# Autodesk Inventor assembly: 右足アセンブリ_MIR
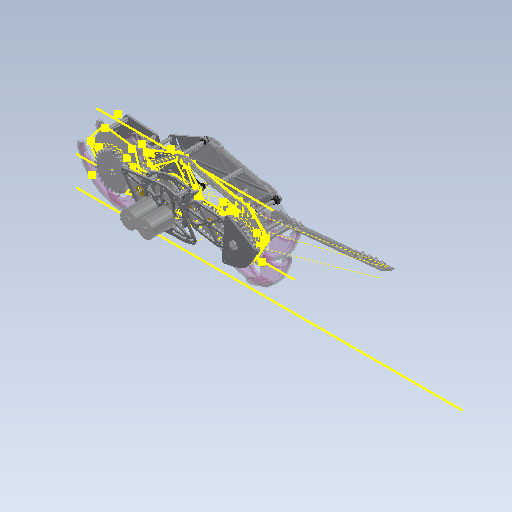
[picture p0: Inventor's stored thumbnail of the model, 512x512]
Saved by Autodesk Inventor 2020 (Build 240168000, 168)
## iProperties
Created: 2019-09-17
Part Number: 右足アセンブリ_MIR
Material: 一般
Document SubType Name: Assembly
Designer: tanjihayato
Mass: 648.248 g
Surface Area: 3194.36 cm^2
Volume: 323.123 cm^3
Density: 2.00619 g/cm^3
Author: tanjihayato
## Documents named in this file (44)
- \\Mac\Home\Documents\Inventor\2019お遊び機体\右足アセンブリ_MIR.iam
- \\Mac\Home\Documents\Inventor\2019お遊び機体\前足内フレーム_MIR1.ipt
- \\Mac\Home\Documents\Inventor\2019お遊び機体\新型３クランクアセンブリ_MIR2.iam
- \\Mac\Home\Documents\Inventor\2019お遊び機体\新型３脚最終段カム.ipt
- \\Mac\Home\Documents\Inventor\2019お遊び機体\スペーサ　m3-l35.ipt
- \\Mac\Home\Documents\Inventor\2019お遊び機体\新型３ヘッケン_MIR2.ipt
- \\Mac\Home\Documents\Inventor\2019お遊び機体\新型３揺動節_MIR2.ipt
- \\Mac\Home\Documents\Inventor\2019お遊び機体\線図_MIR.ipt
- \\Mac\Home\Documents\Inventor\2019お遊び機体\ギアトレイン_MIR1.ipt
- \\Mac\Home\Documents\Inventor\2019お遊び機体\スペーサ　m3-l6.ipt
- \\Mac\Home\Documents\Inventor\2019お遊び機体\前足外フレーム_MIR1.ipt
- \\Mac\Home\Documents\Inventor\2019お遊び機体\後ろ脚内フレーム_MIR1.ipt
- \\Mac\Home\Documents\Inventor\2019お遊び機体\後ろ脚内フレーム２_MIR1.ipt
- \\Mac\Home\Documents\Inventor\2019お遊び機体\新型３クランクアセンブリ_MIR_MIR1.iam
- \\Mac\Home\Documents\Inventor\2019お遊び機体\新型３ヘッケン_MIR_MIR1.ipt
- \\Mac\Home\Documents\Inventor\2019お遊び機体\新型３揺動節_MIR_MIR1.ipt
- \\Mac\Home\Documents\Inventor\2019お遊び機体\後ろ脚外フレーム_MIR1.ipt
- \\Mac\Home\Documents\Inventor\2019お遊び機体\前足ギアトレイン抑え_MIR.ipt
- \\Mac\Home\Documents\Inventor\2019お遊び機体\スペーサ　m3-l12.ipt
- \\Mac\Home\Documents\Inventor\2019お遊び機体\新型３脚最終段カム2.ipt
- \\Mac\Home\Documents\Inventor\2019お遊び機体\z28ギア(インベンター).ipt
- \\Mac\Home\Documents\Inventor\2019お遊び機体\z20ギア(インベンター).ipt
- \\Mac\Home\Documents\Inventor\2019お遊び機体\ベアリングフランジ6-12.ipt
- \\Mac\Home\Documents\Inventor\2019お遊び機体\z17ギア(インベンター).ipt
- \\Mac\Home\Documents\Inventor\2019お遊び機体\中間内フレーム2_MIR.ipt
- \\Mac\Home\Documents\Inventor\2019お遊び機体\サス軸抑え外_MIR.ipt
- \\Mac\Home\Documents\Inventor\2019お遊び機体\中間外フレーム2_MIR.ipt
- \\Mac\Home\Documents\Inventor\2019お遊び機体\スペーサ　m3-l3.ipt
- \\Mac\Home\Documents\Inventor\2019お遊び機体\タミヤダンパー1.iam
- \\Mac\Home\Documents\Inventor\2019お遊び機体\脚ゴム_MIR.ipt
- \\Mac\Home\Documents\Inventor\2019お遊び機体\歯車m0.5.z80.ipt
- \\Mac\Home\Documents\Inventor\2019お遊び機体\m2z10.ipt
- \\Mac\Home\Documents\Inventor\2019お遊び機体\中間フレーム内内_MIR.ipt
- \\Mac\Home\Documents\Inventor\2019お遊び機体\モーター(形だけ).ipt
- \\Mac\Home\Documents\Inventor\2019お遊び機体\スペーサ　m3-l20.ipt
- \\Mac\Home\Documents\Inventor\2019お遊び機体\脚モーターマウント_MIR.ipt
- \\Mac\Home\Documents\Inventor\2019お遊び機体\台形サスバー２.ipt
- \\Mac\Home\Documents\Inventor\2019お遊び機体\フランジブッシュ　d6-D8-l5-h12.ipt
- \\Mac\Home\Documents\Inventor\2019お遊び機体\スペーサ　m3-l45.ipt
- \\Mac\Home\Documents\Inventor\2019お遊び機体\台形サスバー板.ipt
- \\Mac\Home\Documents\Inventor\2019お遊び機体\台形サスカバー_MIR.ipt
- \\Mac\Home\Documents\Inventor\2019お遊び機体\カウンター短.ipt
- \\Mac\Home\Documents\Inventor\2019お遊び機体\ベアリングH　d6-D10-B3.ipt
- \\Mac\Home\Documents\Inventor\2019お遊び機体\スペーサ　m4-l35.ipt
## Components (114 placed, 43 different names)
1. 前足内フレーム_MIR1:1 — 挿入:29, 挿入:32, 挿入:37, 挿入:59, 挿入:61, 挿入:126, 挿入:127, 挿入:135, 挿入:134, 挿入:107, 挿入:108
2. 新型３クランクアセンブリ_MIR2:1 [sub-assembly] — メイト:1, 挿入:1, 挿入:11, 挿入:10, 挿入:9, 挿入:8
3. 新型３脚最終段カム:1 — メイト:1, 挿入:1, メイト:44, 挿入:62, 挿入:107
4. スペーサ　m3-l35:1 — 挿入:29
5. スペーサ　m3-l35:2 — 挿入:32, メイト:2, メイト:3, メイト:4, メイト:5, メイト:15
6. 新型３ヘッケン_MIR2:1 — 挿入:11, 挿入:14, フラッシュ:2, メイト:57, メイト:56
7. 新型３ヘッケン_MIR2:2 — 挿入:10, 挿入:13, フラッシュ:4, メイト:61, メイト:60
8. 新型３ヘッケン_MIR2:3 — 挿入:9, 挿入:12, フラッシュ:5, メイト:63, メイト:62
9. 新型３ヘッケン_MIR2:4 — 挿入:8, 挿入:7, フラッシュ:3, メイト:59, メイト:58
10. 新型３揺動節_MIR2:1 — 挿入:7, メイト:2
11. 新型３揺動節_MIR2:2 — 挿入:13, メイト:3
12. 新型３揺動節_MIR2:3 — 挿入:12, メイト:4
13. 新型３揺動節_MIR2:4 — 挿入:14, メイト:5
14. 線図_MIR:1 — メイト:51
15. ギアトレイン_MIR1:1 — 挿入:17, 挿入:20, 挿入:19, 挿入:16, 挿入:15, 挿入:18, 挿入:103
16. ギアトレイン_MIR1:2 — 挿入:37, メイト:10, 挿入:21
17. スペーサ　m3-l6:1 — 挿入:17
18. スペーサ　m3-l6:2 — メイト:10, 挿入:20
19. スペーサ　m3-l6:3 — 挿入:19
20. スペーサ　m3-l6:4 — 挿入:16, 挿入:69
21. スペーサ　m3-l6:5 — 挿入:21, 挿入:15
22. スペーサ　m3-l6:6 — 挿入:18, 挿入:67
23. スペーサ　m3-l35:3 — 挿入:119, 挿入:84, メイト:55
24. スペーサ　m3-l35:4 — 挿入:82
25. スペーサ　m3-l35:5 — メイト:53, 挿入:83
26. 前足外フレーム_MIR1:1 — メイト:15, 挿入:125, 挿入:128, メイト:84, 挿入:136, 挿入:105
27. 後ろ脚内フレーム_MIR1:1 — メイト:17, 挿入:41, 挿入:71, 挿入:73, 挿入:76, 挿入:77
28. 後ろ脚内フレーム２_MIR1:1 — メイト:17, 挿入:41, 挿入:52, 挿入:51, 挿入:54, 挿入:53, 挿入:106
29. 新型３クランクアセンブリ_MIR_MIR1:1 [sub-assembly] — 挿入:43, 挿入:44, 挿入:45, 挿入:46, メイト:18, 挿入:55
30. 新型３ヘッケン_MIR_MIR1:1 — 挿入:43, 挿入:50, フラッシュ:7, メイト:67, メイト:66
31. 新型３ヘッケン_MIR_MIR1:2 — 挿入:44, 挿入:48, フラッシュ:6, メイト:65, メイト:64
32. 新型３ヘッケン_MIR_MIR1:3 — 挿入:45, 挿入:49, フラッシュ:8, メイト:69, メイト:68
33. 新型３ヘッケン_MIR_MIR1:4 — 挿入:46, 挿入:47, フラッシュ:9, メイト:71, メイト:70
34. 新型３揺動節_MIR_MIR1:1 — 挿入:47, メイト:20
35. 新型３揺動節_MIR_MIR1:2 — 挿入:48, メイト:22
36. 新型３揺動節_MIR_MIR1:3 — 挿入:49, メイト:21
37. 新型３揺動節_MIR_MIR1:4 — 挿入:50, メイト:19
38. スペーサ　m3-l35:6 — 挿入:52, メイト:23
39. スペーサ　m3-l35:7 — 挿入:51
40. スペーサ　m3-l35:8 — メイト:22, メイト:21, メイト:20, メイト:19, 挿入:54, 挿入:57
41. スペーサ　m3-l35:9 — 挿入:53
42. 新型３脚最終段カム:2 — メイト:18, 挿入:55, メイト:48, 挿入:74, 挿入:106
43. 後ろ脚外フレーム_MIR1:1 — メイト:23, 挿入:57, 挿入:104
44. 前足ギアトレイン抑え_MIR:1 — 挿入:109, メイト:53
45. スペーサ　m3-l12:1 — 挿入:61, メイト:53
46. スペーサ　m3-l12:2 — 挿入:59
47. スペーサ　m3-l12:3 — 挿入:108, 挿入:109
48. 新型３脚最終段カム2:1 — メイト:44, 挿入:62, メイト:45, 挿入:63
49. z28ギア(インベンター):1 — メイト:45, 挿入:63, メイト:47, 挿入:64
50. 新型３脚最終段カム:3 — メイト:46, 挿入:65
51. 新型３脚最終段カム:4 — メイト:47, メイト:46, 挿入:65, 挿入:64
52. z20ギア(インベンター):1 — 挿入:66
53. ベアリングフランジ6-12:1 — 挿入:67, 挿入:66
54. z17ギア(インベンター):1 — 挿入:68
55. ベアリングフランジ6-12:2 — 挿入:69, 挿入:68
56. z17ギア(インベンター):2 — 挿入:70
57. ベアリングフランジ6-12:3 — 挿入:71, 挿入:70
58. z20ギア(インベンター):2 — 挿入:72
59. ベアリングフランジ6-12:4 — 挿入:73, 挿入:72
60. z28ギア(インベンター):2 — メイト:49, 挿入:75
61. 新型３脚最終段カム:5 — メイト:49, 挿入:75, メイト:48, 挿入:74
62. スペーサ　m3-l6:7 — 挿入:76, メイト:52
63. スペーサ　m3-l6:8 — 挿入:77
64. 中間内フレーム2_MIR:1 — メイト:51, メイト:50, 挿入:78, 挿入:86, 挿入:88, 挿入:85, 挿入:94, 挿入:98, 挿入:96, 挿入:95, 挿入:97, 挿入:124
65. サス軸抑え外_MIR:1 — メイト:50, 挿入:78
66. 中間外フレーム2_MIR:1 — 挿入:119, メイト:53, メイト:79, 挿入:120
67. スペーサ　m3-l3:1 — 挿入:86, 挿入:82
68. スペーサ　m3-l3:2 — 挿入:88, 挿入:84
69. スペーサ　m3-l3:3 — 挿入:85, 挿入:83
70. タミヤダンパー1:1 [sub-assembly] — メイト:55, 挿入:118
71. 脚ゴム_MIR:1 — フラッシュ:8, メイト:69, メイト:68
72. 脚ゴム_MIR:2 — フラッシュ:9, メイト:71, メイト:70
73. 脚ゴム_MIR:3 — フラッシュ:2, メイト:57, メイト:56
74. 脚ゴム_MIR:4 — フラッシュ:7, メイト:67, メイト:66
75. 脚ゴム_MIR:5 — フラッシュ:4, メイト:61, メイト:60
76. 脚ゴム_MIR:6 — フラッシュ:6, メイト:65, メイト:64
77. 脚ゴム_MIR:7 — フラッシュ:5, メイト:63, メイト:62
78. 脚ゴム_MIR:8 — フラッシュ:3, メイト:59, メイト:58
79. 歯車m0.5.z80:1 — メイト:74, 挿入:105, 挿入:104, 挿入:103, 挿入:102
80. m2z10:1 — メイト:74, 挿入:94, 挿入:106
81. スペーサ　m3-l6:9 — 挿入:98, メイト:73, メイト:75
82. スペーサ　m3-l6:10 — 挿入:96
83. スペーサ　m3-l6:11 — 挿入:95
84. スペーサ　m3-l6:12 — 挿入:97, 挿入:99, 挿入:107
85. サス軸抑え外_MIR:2 — メイト:73, 挿入:99, メイト:52, 挿入:103
86. スペーサ　m3-l6:13 — 挿入:105
87. スペーサ　m3-l6:14 — 挿入:104
88. スペーサ　m3-l6:15 — 挿入:103
89. スペーサ　m3-l6:16 — 挿入:106, 挿入:102
90. 中間フレーム内内_MIR:1 — メイト:75, 挿入:107, 挿入:108, 挿入:111, 挿入:110, 挿入:109
91. モーター(形だけ):1
92. モーター(形だけ):2
93. スペーサ　m3-l20:1 — 挿入:108, 挿入:112
94. スペーサ　m3-l20:2 — 挿入:111
95. スペーサ　m3-l20:3 — 挿入:110
96. スペーサ　m3-l20:4 — 挿入:109, メイト:76
97. 脚モーターマウント_MIR:1 — メイト:76, 挿入:112
98. 台形サスバー２:1 — 挿入:125, メイト:79, 挿入:121, 挿入:122, 挿入:123, 挿入:129, メイト:83, 挿入:130
99. 台形サスバー２:2 — 挿入:126, 挿入:118, メイト:80, メイト:82, フラッシュ:10, メイト:81
100. フランジブッシュ　d6-D8-l5-h12:1 — 挿入:128
101. フランジブッシュ　d6-D8-l5-h12:2 — 挿入:120
102. フランジブッシュ　d6-D8-l5-h12:3 — 挿入:127
103. フランジブッシュ　d6-D8-l5-h12:4 — 挿入:124
104. スペーサ　m3-l45:1 — メイト:80, 挿入:121
105. スペーサ　m3-l45:2 — 挿入:122
106. スペーサ　m3-l45:3 — 挿入:123
107. スペーサ　m3-l45:4 — 挿入:129
108. 台形サスバー板:1 — メイト:82, フラッシュ:10, メイト:81
109. 台形サスカバー_MIR:1 — メイト:83, 挿入:130
110. カウンター短:1 — メイト:84, 挿入:136
111. ベアリングH　d6-D10-B3:1 — 挿入:104
112. ベアリングH　d6-D10-B3:2 — 挿入:105
113. スペーサ　m4-l35:1 — 挿入:135
114. スペーサ　m4-l35:2 — 挿入:134
## Relationships (160: Insert 99, Mate 52, Flush 9)
- メイト:1 [Mate]: 新型３クランクアセンブリ_MIR2:1 ↔ 新型３脚最終段カム:1
- 挿入:1 [Insert]: 新型３クランクアセンブリ_MIR2:1 ↔ 新型３脚最終段カム:1
- 挿入:29 [Insert]: 前足内フレーム_MIR1:1 ↔ スペーサ　m3-l35:1
- 挿入:32 [Insert]: 前足内フレーム_MIR1:1 ↔ スペーサ　m3-l35:2
- 挿入:11 [Insert] (0.25 mm): 新型３クランクアセンブリ_MIR2:1 ↔ 新型３ヘッケン_MIR2:1
- 挿入:10 [Insert] (0.25 mm): 新型３クランクアセンブリ_MIR2:1 ↔ 新型３ヘッケン_MIR2:2
- 挿入:9 [Insert] (0.25 mm): 新型３クランクアセンブリ_MIR2:1 ↔ 新型３ヘッケン_MIR2:3
- 挿入:8 [Insert] (0.25 mm): 新型３クランクアセンブリ_MIR2:1 ↔ 新型３ヘッケン_MIR2:4
- 挿入:7 [Insert]: 新型３ヘッケン_MIR2:4 ↔ 新型３揺動節_MIR2:1
- メイト:2 [Mate]: スペーサ　m3-l35:2 ↔ 新型３揺動節_MIR2:1
- 挿入:13 [Insert]: 新型３ヘッケン_MIR2:2 ↔ 新型３揺動節_MIR2:2
- メイト:3 [Mate]: スペーサ　m3-l35:2 ↔ 新型３揺動節_MIR2:2
- 挿入:12 [Insert]: 新型３ヘッケン_MIR2:3 ↔ 新型３揺動節_MIR2:3
- メイト:4 [Mate]: スペーサ　m3-l35:2 ↔ 新型３揺動節_MIR2:3
- 挿入:14 [Insert]: 新型３ヘッケン_MIR2:1 ↔ 新型３揺動節_MIR2:4
- メイト:5 [Mate]: スペーサ　m3-l35:2 ↔ 新型３揺動節_MIR2:4
- 挿入:37 [Insert]: 前足内フレーム_MIR1:1 ↔ ギアトレイン_MIR1:2
- 挿入:17 [Insert]: ギアトレイン_MIR1:1 ↔ スペーサ　m3-l6:1
- メイト:10 [Mate]: ギアトレイン_MIR1:2 ↔ スペーサ　m3-l6:2
- 挿入:20 [Insert]: ギアトレイン_MIR1:1 ↔ スペーサ　m3-l6:2
- 挿入:19 [Insert]: ギアトレイン_MIR1:1 ↔ スペーサ　m3-l6:3
- 挿入:16 [Insert]: ギアトレイン_MIR1:1 ↔ スペーサ　m3-l6:4
- 挿入:21 [Insert]: ギアトレイン_MIR1:2 ↔ スペーサ　m3-l6:5
- 挿入:15 [Insert]: ギアトレイン_MIR1:1 ↔ スペーサ　m3-l6:5
- 挿入:18 [Insert]: ギアトレイン_MIR1:1 ↔ スペーサ　m3-l6:6
- メイト:15 [Mate]: スペーサ　m3-l35:2 ↔ 前足外フレーム_MIR1:1
- メイト:17 [Mate]: 後ろ脚内フレーム_MIR1:1 ↔ 後ろ脚内フレーム２_MIR1:1
- 挿入:41 [Insert]: 後ろ脚内フレーム_MIR1:1 ↔ 後ろ脚内フレーム２_MIR1:1
- 挿入:43 [Insert] (0.25 mm): 新型３クランクアセンブリ_MIR_MIR1:1 ↔ 新型３ヘッケン_MIR_MIR1:1
- 挿入:44 [Insert] (0.25 mm): 新型３クランクアセンブリ_MIR_MIR1:1 ↔ 新型３ヘッケン_MIR_MIR1:2
- 挿入:45 [Insert] (0.25 mm): 新型３クランクアセンブリ_MIR_MIR1:1 ↔ 新型３ヘッケン_MIR_MIR1:3
- 挿入:46 [Insert] (0.25 mm): 新型３クランクアセンブリ_MIR_MIR1:1 ↔ 新型３ヘッケン_MIR_MIR1:4
- 挿入:47 [Insert]: 新型３ヘッケン_MIR_MIR1:4 ↔ 新型３揺動節_MIR_MIR1:1
- 挿入:48 [Insert]: 新型３ヘッケン_MIR_MIR1:2 ↔ 新型３揺動節_MIR_MIR1:2
- 挿入:49 [Insert]: 新型３ヘッケン_MIR_MIR1:3 ↔ 新型３揺動節_MIR_MIR1:3
- 挿入:50 [Insert]: 新型３ヘッケン_MIR_MIR1:1 ↔ 新型３揺動節_MIR_MIR1:4
- 挿入:52 [Insert]: 後ろ脚内フレーム２_MIR1:1 ↔ スペーサ　m3-l35:6
- 挿入:51 [Insert]: 後ろ脚内フレーム２_MIR1:1 ↔ スペーサ　m3-l35:7
- メイト:22 [Mate]: 新型３揺動節_MIR_MIR1:2 ↔ スペーサ　m3-l35:8
- メイト:21 [Mate]: 新型３揺動節_MIR_MIR1:3 ↔ スペーサ　m3-l35:8
- メイト:20 [Mate]: 新型３揺動節_MIR_MIR1:1 ↔ スペーサ　m3-l35:8
- メイト:19 [Mate]: 新型３揺動節_MIR_MIR1:4 ↔ スペーサ　m3-l35:8
- 挿入:54 [Insert]: 後ろ脚内フレーム２_MIR1:1 ↔ スペーサ　m3-l35:8
- 挿入:53 [Insert]: 後ろ脚内フレーム２_MIR1:1 ↔ スペーサ　m3-l35:9
- メイト:18 [Mate]: 新型３クランクアセンブリ_MIR_MIR1:1 ↔ 新型３脚最終段カム:2
- 挿入:55 [Insert]: 新型３クランクアセンブリ_MIR_MIR1:1 ↔ 新型３脚最終段カム:2
- メイト:23 [Mate]: スペーサ　m3-l35:6 ↔ 後ろ脚外フレーム_MIR1:1
- 挿入:57 [Insert]: スペーサ　m3-l35:8 ↔ 後ろ脚外フレーム_MIR1:1
- メイト:44 [Mate]: 新型３脚最終段カム:1 ↔ 新型３脚最終段カム2:1
- 挿入:62 [Insert]: 新型３脚最終段カム:1 ↔ 新型３脚最終段カム2:1
- メイト:45 [Mate]: 新型３脚最終段カム2:1 ↔ z28ギア(インベンター):1
- 挿入:63 [Insert]: 新型３脚最終段カム2:1 ↔ z28ギア(インベンター):1
- メイト:47 [Mate]: z28ギア(インベンター):1 ↔ 新型３脚最終段カム:4
- メイト:46 [Mate]: 新型３脚最終段カム:3 ↔ 新型３脚最終段カム:4
- 挿入:65 [Insert]: 新型３脚最終段カム:3 ↔ 新型３脚最終段カム:4
- 挿入:64 [Insert]: z28ギア(インベンター):1 ↔ 新型３脚最終段カム:4
- 挿入:67 [Insert] (1 mm): スペーサ　m3-l6:6 ↔ ベアリングフランジ6-12:1
- 挿入:66 [Insert]: z20ギア(インベンター):1 ↔ ベアリングフランジ6-12:1
- 挿入:69 [Insert] (1 mm): スペーサ　m3-l6:4 ↔ ベアリングフランジ6-12:2
- 挿入:68 [Insert]: z17ギア(インベンター):1 ↔ ベアリングフランジ6-12:2
- 挿入:71 [Insert] (1 mm): 後ろ脚内フレーム_MIR1:1 ↔ ベアリングフランジ6-12:3
- 挿入:70 [Insert]: z17ギア(インベンター):2 ↔ ベアリングフランジ6-12:3
- 挿入:73 [Insert] (1 mm): 後ろ脚内フレーム_MIR1:1 ↔ ベアリングフランジ6-12:4
- 挿入:72 [Insert]: z20ギア(インベンター):2 ↔ ベアリングフランジ6-12:4
- メイト:49 [Mate]: z28ギア(インベンター):2 ↔ 新型３脚最終段カム:5
- 挿入:75 [Insert]: z28ギア(インベンター):2 ↔ 新型３脚最終段カム:5
- メイト:48 [Mate]: 新型３脚最終段カム:2 ↔ 新型３脚最終段カム:5
- 挿入:74 [Insert]: 新型３脚最終段カム:2 ↔ 新型３脚最終段カム:5
- 挿入:59 [Insert]: 前足内フレーム_MIR1:1 ↔ スペーサ　m3-l12:2
- 挿入:61 [Insert]: 前足内フレーム_MIR1:1 ↔ スペーサ　m3-l12:1
- 挿入:76 [Insert]: 後ろ脚内フレーム_MIR1:1 ↔ スペーサ　m3-l6:7
- 挿入:77 [Insert]: 後ろ脚内フレーム_MIR1:1 ↔ スペーサ　m3-l6:8
- メイト:51 [Mate]: 線図_MIR:1 ↔ 中間内フレーム2_MIR:1
- メイト:50 [Mate]: 中間内フレーム2_MIR:1 ↔ サス軸抑え外_MIR:1
- 挿入:78 [Insert] (1 mm): 中間内フレーム2_MIR:1 ↔ サス軸抑え外_MIR:1
- 挿入:119 [Insert]: スペーサ　m3-l35:3 ↔ 中間外フレーム2_MIR:1
- メイト:53 [Mate]: スペーサ　m3-l35:5 ↔ 中間外フレーム2_MIR:1
- 挿入:86 [Insert]: 中間内フレーム2_MIR:1 ↔ スペーサ　m3-l3:1
- 挿入:82 [Insert]: スペーサ　m3-l35:4 ↔ スペーサ　m3-l3:1
- 挿入:88 [Insert]: 中間内フレーム2_MIR:1 ↔ スペーサ　m3-l3:2
- 挿入:84 [Insert]: スペーサ　m3-l35:3 ↔ スペーサ　m3-l3:2
- 挿入:85 [Insert]: 中間内フレーム2_MIR:1 ↔ スペーサ　m3-l3:3
- 挿入:83 [Insert]: スペーサ　m3-l35:5 ↔ スペーサ　m3-l3:3
- メイト:55 [Mate]: スペーサ　m3-l35:3 ↔ タミヤダンパー1:1
- フラッシュ:8 [Flush]: 新型３ヘッケン_MIR_MIR1:3 ↔ 脚ゴム_MIR:1
- メイト:69 [Mate]: 新型３ヘッケン_MIR_MIR1:3 ↔ 脚ゴム_MIR:1
- メイト:68 [Mate]: 新型３ヘッケン_MIR_MIR1:3 ↔ 脚ゴム_MIR:1
- フラッシュ:9 [Flush]: 新型３ヘッケン_MIR_MIR1:4 ↔ 脚ゴム_MIR:2
- メイト:71 [Mate]: 新型３ヘッケン_MIR_MIR1:4 ↔ 脚ゴム_MIR:2
- メイト:70 [Mate]: 新型３ヘッケン_MIR_MIR1:4 ↔ 脚ゴム_MIR:2
- フラッシュ:2 [Flush]: 新型３ヘッケン_MIR2:1 ↔ 脚ゴム_MIR:3
- メイト:57 [Mate]: 新型３ヘッケン_MIR2:1 ↔ 脚ゴム_MIR:3
- メイト:56 [Mate]: 新型３ヘッケン_MIR2:1 ↔ 脚ゴム_MIR:3
- フラッシュ:7 [Flush]: 新型３ヘッケン_MIR_MIR1:1 ↔ 脚ゴム_MIR:4
- メイト:67 [Mate]: 新型３ヘッケン_MIR_MIR1:1 ↔ 脚ゴム_MIR:4
- メイト:66 [Mate]: 新型３ヘッケン_MIR_MIR1:1 ↔ 脚ゴム_MIR:4
- フラッシュ:4 [Flush]: 新型３ヘッケン_MIR2:2 ↔ 脚ゴム_MIR:5
- メイト:61 [Mate]: 新型３ヘッケン_MIR2:2 ↔ 脚ゴム_MIR:5
- メイト:60 [Mate]: 新型３ヘッケン_MIR2:2 ↔ 脚ゴム_MIR:5
- フラッシュ:6 [Flush]: 新型３ヘッケン_MIR_MIR1:2 ↔ 脚ゴム_MIR:6
- メイト:65 [Mate]: 新型３ヘッケン_MIR_MIR1:2 ↔ 脚ゴム_MIR:6
- メイト:64 [Mate]: 新型３ヘッケン_MIR_MIR1:2 ↔ 脚ゴム_MIR:6
- フラッシュ:5 [Flush]: 新型３ヘッケン_MIR2:3 ↔ 脚ゴム_MIR:7
- メイト:63 [Mate]: 新型３ヘッケン_MIR2:3 ↔ 脚ゴム_MIR:7
- メイト:62 [Mate]: 新型３ヘッケン_MIR2:3 ↔ 脚ゴム_MIR:7
- フラッシュ:3 [Flush]: 新型３ヘッケン_MIR2:4 ↔ 脚ゴム_MIR:8
- メイト:59 [Mate]: 新型３ヘッケン_MIR2:4 ↔ 脚ゴム_MIR:8
- メイト:58 [Mate]: 新型３ヘッケン_MIR2:4 ↔ 脚ゴム_MIR:8
- メイト:74 [Mate]: 歯車m0.5.z80:1 ↔ m2z10:1
- 挿入:94 [Insert] (0.5 mm): 中間内フレーム2_MIR:1 ↔ m2z10:1
- 挿入:98 [Insert]: 中間内フレーム2_MIR:1 ↔ スペーサ　m3-l6:9
- 挿入:96 [Insert]: 中間内フレーム2_MIR:1 ↔ スペーサ　m3-l6:10
- 挿入:95 [Insert]: 中間内フレーム2_MIR:1 ↔ スペーサ　m3-l6:11
- 挿入:97 [Insert]: 中間内フレーム2_MIR:1 ↔ スペーサ　m3-l6:12
- メイト:73 [Mate]: スペーサ　m3-l6:9 ↔ サス軸抑え外_MIR:2
- 挿入:99 [Insert] (4 mm): スペーサ　m3-l6:12 ↔ サス軸抑え外_MIR:2
- 挿入:105 [Insert]: 歯車m0.5.z80:1 ↔ スペーサ　m3-l6:13
- 挿入:104 [Insert]: 歯車m0.5.z80:1 ↔ スペーサ　m3-l6:14
- 挿入:103 [Insert]: 歯車m0.5.z80:1 ↔ スペーサ　m3-l6:15
- 挿入:106 [Insert]: m2z10:1 ↔ スペーサ　m3-l6:16
- 挿入:102 [Insert]: 歯車m0.5.z80:1 ↔ スペーサ　m3-l6:16
- メイト:75 [Mate]: スペーサ　m3-l6:9 ↔ 中間フレーム内内_MIR:1
- 挿入:107 [Insert]: スペーサ　m3-l6:12 ↔ 中間フレーム内内_MIR:1
- 挿入:108 [Insert]: 中間フレーム内内_MIR:1 ↔ スペーサ　m3-l20:1
- 挿入:111 [Insert]: 中間フレーム内内_MIR:1 ↔ スペーサ　m3-l20:2
- 挿入:110 [Insert]: 中間フレーム内内_MIR:1 ↔ スペーサ　m3-l20:3
- 挿入:109 [Insert]: 中間フレーム内内_MIR:1 ↔ スペーサ　m3-l20:4
- メイト:76 [Mate]: スペーサ　m3-l20:4 ↔ 脚モーターマウント_MIR:1
- 挿入:112 [Insert] (-2 mm): スペーサ　m3-l20:1 ↔ 脚モーターマウント_MIR:1
- 挿入:125 [Insert] (1 mm): 前足外フレーム_MIR1:1 ↔ 台形サスバー２:1
- メイト:79 [Mate]: 中間外フレーム2_MIR:1 ↔ 台形サスバー２:1
- 挿入:126 [Insert] (4 mm): 前足内フレーム_MIR1:1 ↔ 台形サスバー２:2
- 挿入:118 [Insert] (15 mm): タミヤダンパー1:1 ↔ 台形サスバー２:2
- 挿入:128 [Insert]: 前足外フレーム_MIR1:1 ↔ フランジブッシュ　d6-D8-l5-h12:1
- 挿入:120 [Insert]: 中間外フレーム2_MIR:1 ↔ フランジブッシュ　d6-D8-l5-h12:2
- 挿入:127 [Insert]: 前足内フレーム_MIR1:1 ↔ フランジブッシュ　d6-D8-l5-h12:3
- 挿入:124 [Insert]: 中間内フレーム2_MIR:1 ↔ フランジブッシュ　d6-D8-l5-h12:4
- メイト:80 [Mate]: 台形サスバー２:2 ↔ スペーサ　m3-l45:1
- 挿入:121 [Insert]: 台形サスバー２:1 ↔ スペーサ　m3-l45:1
- 挿入:122 [Insert]: 台形サスバー２:1 ↔ スペーサ　m3-l45:2
- 挿入:123 [Insert]: 台形サスバー２:1 ↔ スペーサ　m3-l45:3
- 挿入:129 [Insert]: 台形サスバー２:1 ↔ スペーサ　m3-l45:4
- メイト:82 [Mate]: 台形サスバー２:2 ↔ 台形サスバー板:1
- フラッシュ:10 [Flush]: 台形サスバー２:2 ↔ 台形サスバー板:1
- メイト:81 [Mate]: 台形サスバー２:2 ↔ 台形サスバー板:1
- メイト:83 [Mate]: 台形サスバー２:1 ↔ 台形サスカバー_MIR:1
- 挿入:130 [Insert]: 台形サスバー２:1 ↔ 台形サスカバー_MIR:1
- メイト:84 [Mate]: 前足外フレーム_MIR1:1 ↔ カウンター短:1
- 挿入:136 [Insert]: 前足外フレーム_MIR1:1 ↔ カウンター短:1
- 挿入:135 [Insert]: 前足内フレーム_MIR1:1 ↔ スペーサ　m4-l35:1
- 挿入:134 [Insert]: 前足内フレーム_MIR1:1 ↔ スペーサ　m4-l35:2
- メイト:52 [Mate]: スペーサ　m3-l6:7 ↔ サス軸抑え外_MIR:2
- 挿入:103 [Insert] (1 mm): ギアトレイン_MIR1:1 ↔ サス軸抑え外_MIR:2
- 挿入:104 [Insert]: 後ろ脚外フレーム_MIR1:1 ↔ ベアリングH　d6-D10-B3:1
- 挿入:105 [Insert]: 前足外フレーム_MIR1:1 ↔ ベアリングH　d6-D10-B3:2
- 挿入:106 [Insert] (-0.5 mm): 後ろ脚内フレーム２_MIR1:1 ↔ 新型３脚最終段カム:2
- 挿入:107 [Insert] (-1 mm): 前足内フレーム_MIR1:1 ↔ 新型３脚最終段カム:1
- 挿入:108 [Insert]: 前足内フレーム_MIR1:1 ↔ スペーサ　m3-l12:3
- 挿入:109 [Insert]: 前足ギアトレイン抑え_MIR:1 ↔ スペーサ　m3-l12:3
- メイト:53 [Mate]: 前足ギアトレイン抑え_MIR:1 ↔ スペーサ　m3-l12:1
